# Autodesk Inventor assembly: ReelAssembly_SBail
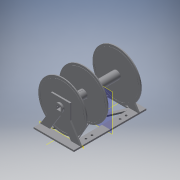
[picture p0: Inventor's stored thumbnail of the model, 180x180]
Saved by Autodesk Inventor 2019 (Build 230136000, 136)
## iProperties
Created: 2019-04-17
Part Number: ReelAssembly_SBail
Document SubType Name: Assembly
Designer: samson.bailor
Author: samson.bailor
## Documents named in this file (5)
- S:\Modern Technology Academy\Bogdziewicz\Student Drop Box\1-Collaboration\47-EDD-2019\Trotline\trotline-reel\src\inventor\ReelAssembly_SBail.iam
- S:\Modern Technology Academy\Bogdziewicz\Student Drop Box\1-Collaboration\47-EDD-2019\Trotline\trotline-reel\src\inventor\Axel_SBail.ipt
- S:\Modern Technology Academy\Bogdziewicz\Student Drop Box\1-Collaboration\47-EDD-2019\Trotline\trotline-reel\src\inventor\Plate.ipt
- S:\Modern Technology Academy\Bogdziewicz\Student Drop Box\1-Collaboration\47-EDD-2019\Trotline\trotline-reel\src\inventor\PlateCenter.ipt
- S:\Modern Technology Academy\Bogdziewicz\Student Drop Box\1-Collaboration\47-EDD-2019\Trotline\trotline-reel\src\inventor\Square Support.ipt
## Components (5 placed, 4 different names)
1. Axel_SBail:1 — Mate:3, Insert:1, Insert:2, Insert:3
2. PlateCenter:1 — Mate:3
3. Plate:3 — Insert:1
4. Plate:4 — Insert:2
5. Square Support:1 — Insert:3
## Relationships (4: Insert 3, Mate 1)
- Mate:3: Axel_SBail:1 ↔ PlateCenter:1
- Insert:1: Axel_SBail:1 ↔ Plate:3
- Insert:2: Axel_SBail:1 ↔ Plate:4
- Insert:3: Axel_SBail:1 ↔ Square Support:1
